# Autodesk Inventor assembly: Joystick
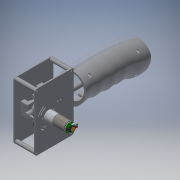
[picture p0: Inventor's stored thumbnail of the model, 180x180]
Saved by Autodesk Inventor 2018 (Build 220112000, 112)
## iProperties
Created: 2019-06-03
Part Number: Joystick
Document SubType Name: Assembly
Designer: aal_9
Author: aal_9
## Documents named in this file (19)
- C:\Users\aal_9\OneDrive\Documentos\Suiza\Courses\Tesis\Joystick\Joystick.iam
- C:\Users\aal_9\OneDrive\Documentos\Suiza\Courses\Tesis\Joystick\SheetConnector.ipt
- C:\Users\aal_9\OneDrive\Documentos\Suiza\Courses\Tesis\Joystick\SheetMotor.ipt
- C:\Users\aal_9\OneDrive\Documentos\Suiza\Courses\Tesis\Joystick\SheetPot.ipt
- C:\Users\aal_9\OneDrive\Documentos\Suiza\Courses\Tesis\Joystick\Spring support.ipt
- C:\Users\aal_9\OneDrive\Documentos\Suiza\Courses\Tesis\Joystick\25d-gearmotor-3d-models\25d-metal-gearmotor-34-47-encoder.ipt
- C:\Users\aal_9\OneDrive\Documentos\Suiza\Courses\Tesis\Joystick\Potentiometer.ipt
- C:\Users\aal_9\OneDrive\Documentos\Suiza\Courses\Tesis\Joystick\MotorPotCouple.ipt
- C:\Users\aal_9\OneDrive\Documentos\Suiza\Courses\Tesis\Joystick\Lever.ipt
- C:\Users\aal_9\OneDrive\Documentos\Suiza\Courses\Tesis\Joystick\RotationShell.ipt
- C:\Users\aal_9\OneDrive\Documentos\Suiza\Courses\Tesis\Joystick\Limit\c-1825043-03-b1-3d.ipt
- C:\Users\aal_9\OneDrive\Documentos\Suiza\Courses\Tesis\Joystick\K-166-Durovis\K-166-Durovis.ipt
- C:\Users\aal_9\OneDrive\Documentos\Suiza\Courses\Tesis\Joystick\Washer.ipt
- C:\Users\aal_9\OneDrive\Documentos\Suiza\Courses\Tesis\Joystick\BarLimitSwitch.ipt
- C:\Users\aal_9\OneDrive\Documentos\Suiza\Courses\Tesis\Joystick\Enconders\3531_0_3D\3531_0.iam
- C:\Users\aal_9\OneDrive\Documentos\Suiza\Courses\Tesis\Joystick\HalfEncoderSupprt.ipt
- C:\Users\aal_9\OneDrive\Documentos\Suiza\Courses\Tesis\Joystick\HandleLeft.ipt
- C:\Users\aal_9\OneDrive\Documentos\Suiza\Courses\Tesis\Joystick\HandleRight.ipt
- C:\Users\aal_9\OneDrive\Documentos\Suiza\Courses\Tesis\Joystick\BF-1209-Durovis\BF-1209-Durovis.iam
## Components (23 placed, 18 different names)
1. SheetConnector:1 — Flush:1, Mate:6
2. SheetMotor:1 — Mate:1, Mate:3, Mate:4, Mate:8, Mate:10, Flush:6, Mate:14, Mate:15, Mate:16, Mate:19, Angle:1, Mate:20, Angle:2, Mate:22, Mate:23, Angle:3
3. SheetPot:1 — Mate:2, Mate:3, Mate:4, Mate:5, Mate:6, Mate:7, Mate:9, Mate:11, Mate:12, Mate:13
4. SheetConnector:2 — Flush:1, Flush:2, Mate:1, Mate:2, Mate:5
5. SheetConnector:3 — Flush:2, Flush:3, Mate:8
6. SheetConnector:4 — Flush:3, Mate:7
7. Spring support:1 — Mate:10, Mate:11, Flush:6, Mate:27
8. 25d-metal-gearmotor-34-47-encoder:1 — Mate:14, Mate:15, Mate:16
9. Potentiometer:1 — Mate:12, Mate:13, Mate:17
10. MotorPotCouple:1 — Mate:17, Mate:18, Mate:19, Flush:7, Mate:21
11. Lever:1 — Mate:18, Angle:1, Flush:7, Mate:24, Mate:25, Mate:26, Flush:8, Mate:36, Mate:37, Angle:4, Mate:40, Mate:47, Angle:5
12. RotationShell:1 — Mate:20, Mate:21, Angle:2, Mate:27
13. c-1825043-03-b1-3d:1 — Mate:22
14. c-1825043-03-b1-3d:2 — Mate:23
15. K-166-Durovis:1
16. Washer:1 — Mate:24, Flush:8, Tangent:1
17. BarLimitSwitch:1 — Mate:25, Mate:26, Angle:3, Angle:5
18. 3531_0:1 [sub-assembly] — Mate:39, Mate:40, Mate:41
19. HalfEncoderSupprt:1 — Mate:34, Mate:35, Mate:36, Flush:9, Mate:41, Mate:43, Mate:44, Mate:46
20. HalfEncoderSupprt:2 — Mate:34, Mate:35, Flush:9, Mate:37, Mate:39, Angle:4, Mate:42
21. HandleLeft:1 — Mate:42, Mate:43, Mate:44, Flush:10, Mate:45
22. HandleRight:1 — Flush:10, Mate:45, Mate:46
23. BF-1209-Durovis:1 [sub-assembly] — Mate:47, Tangent:1
## Relationships (54: Mate 40, Flush 8, Angle 5, Tangent 1)
- Flush:1: SheetConnector:1 ↔ SheetConnector:2
- Flush:2: SheetConnector:2 ↔ SheetConnector:3
- Flush:3: SheetConnector:3 ↔ SheetConnector:4
- Mate:1: SheetMotor:1 ↔ SheetConnector:2
- Mate:2: SheetPot:1 ↔ SheetConnector:2
- Mate:3: SheetMotor:1 ↔ SheetPot:1
- Mate:4: SheetMotor:1 ↔ SheetPot:1
- Mate:5: SheetPot:1 ↔ SheetConnector:2
- Mate:6: SheetConnector:1 ↔ SheetPot:1
- Mate:7: SheetPot:1 ↔ SheetConnector:4
- Mate:8: SheetMotor:1 ↔ SheetConnector:3
- Mate:9: SheetPot:1
- Mate:10: SheetMotor:1 ↔ Spring support:1
- Mate:11: SheetPot:1 ↔ Spring support:1
- Flush:6 (45 mm): SheetMotor:1 ↔ Spring support:1
- Mate:12: SheetPot:1 ↔ Potentiometer:1
- Mate:13: SheetPot:1 ↔ Potentiometer:1
- Mate:14: SheetMotor:1 ↔ 25d-metal-gearmotor-34-47-encoder:1
- Mate:15: SheetMotor:1 ↔ 25d-metal-gearmotor-34-47-encoder:1
- Mate:16: SheetMotor:1 ↔ 25d-metal-gearmotor-34-47-encoder:1
- Mate:17: Potentiometer:1 ↔ MotorPotCouple:1
- Mate:18: MotorPotCouple:1 ↔ Lever:1
- Mate:19 (1 mm): SheetMotor:1 ↔ MotorPotCouple:1
- Angle:1 (90 deg): SheetMotor:1 ↔ Lever:1
- Flush:7 (-30 mm): MotorPotCouple:1 ↔ Lever:1
- Mate:20: SheetMotor:1 ↔ RotationShell:1
- Mate:21: MotorPotCouple:1 ↔ RotationShell:1
- Angle:2 (0 deg): SheetMotor:1 ↔ RotationShell:1
- Mate:22: SheetMotor:1 ↔ c-1825043-03-b1-3d:1
- Mate:23: SheetMotor:1 ↔ c-1825043-03-b1-3d:2
- Mate:24: Lever:1 ↔ Washer:1
- Mate:25: Lever:1 ↔ BarLimitSwitch:1
- Mate:26: Lever:1 ↔ BarLimitSwitch:1
- Angle:3 (180 deg): SheetMotor:1 ↔ BarLimitSwitch:1
- Flush:8: Lever:1 ↔ Washer:1
- Mate:27 (3 mm): Spring support:1 ↔ RotationShell:1
- Mate:34: HalfEncoderSupprt:1 ↔ HalfEncoderSupprt:2
- Mate:35: HalfEncoderSupprt:1 ↔ HalfEncoderSupprt:2
- Mate:36: Lever:1 ↔ HalfEncoderSupprt:1
- Flush:9: HalfEncoderSupprt:1 ↔ HalfEncoderSupprt:2
- Mate:37: Lever:1 ↔ HalfEncoderSupprt:2
- Mate:39: 3531_0:1 ↔ HalfEncoderSupprt:2
- Angle:4 (35 deg): Lever:1 ↔ HalfEncoderSupprt:2
- Mate:40: Lever:1 ↔ 3531_0:1
- Mate:41: 3531_0:1 ↔ HalfEncoderSupprt:1
- Mate:42: HalfEncoderSupprt:2 ↔ HandleLeft:1
- Mate:43: HalfEncoderSupprt:1 ↔ HandleLeft:1
- Mate:44: HalfEncoderSupprt:1 ↔ HandleLeft:1
- Flush:10: HandleLeft:1 ↔ HandleRight:1
- Mate:45: HandleLeft:1 ↔ HandleRight:1
- Mate:46: HalfEncoderSupprt:1 ↔ HandleRight:1
- Mate:47: Lever:1 ↔ BF-1209-Durovis:1
- Tangent:1: Washer:1 ↔ BF-1209-Durovis:1
- Angle:5 (0 deg): Lever:1 ↔ BarLimitSwitch:1
